# Autodesk Inventor assembly: Assembly1
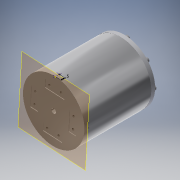
[picture p0: Inventor's stored thumbnail of the model, 180x180]
Saved by Autodesk Inventor 2017 (Build 210142000, 142)
## iProperties
Created: 2016-07-05
Part Number: Assembly1
Document SubType Name: Assembly
Designer: Andres
Author: Andres
## Documents named in this file (6)
- \\Mac\Home\Documents\repositorios\BoreholeCamera\CAD_Probe\Enclosure\Assembly\Assembly1.iam
- \\Mac\Home\Documents\repositorios\BoreholeCamera\CAD_Probe\Enclosure\Parts\Enclosure.ipt
- \\Mac\Home\Documents\repositorios\BoreholeCamera\CAD_Probe\Enclosure\Parts\TYPE 316 SS SOCKET HEAD CAP SCREW.ipt
- \\Mac\Home\Documents\repositorios\BoreholeCamera\CAD_Probe\Enclosure\Parts\SealCover.ipt
- \\Mac\Home\Documents\repositorios\BoreholeCamera\CAD_Probe\Enclosure\Assembly\Assembly1\Design Accelerator\O-Ring3.iam
- \\Mac\Home\Documents\repositorios\BoreholeCamera\CAD_Probe\Enclosure\Assembly\Cover.iam
## Components (13 placed, 5 different names)
1. Enclosure:1 — Rigid:1, Rigid:2, Mate:1, Mate:2, Rigid:3
2. Cover:2 [sub-assembly] — Rigid:3
3. TYPE 316 SS SOCKET HEAD CAP SCREW:2
4. TYPE 316 SS SOCKET HEAD CAP SCREW:4
5. TYPE 316 SS SOCKET HEAD CAP SCREW:6
6. TYPE 316 SS SOCKET HEAD CAP SCREW:7
7. TYPE 316 SS SOCKET HEAD CAP SCREW:8
8. TYPE 316 SS SOCKET HEAD CAP SCREW:9
9. TYPE 316 SS SOCKET HEAD CAP SCREW:11
10. TYPE 316 SS SOCKET HEAD CAP SCREW:12
11. SealCover:1 — Rigid:1
12. SealCover:2 — Rigid:2
13. O-Ring:1 [sub-assembly] — Mate:1, Mate:2
## Relationships (5: WeldJoint 3, Mate 2)
- Rigid:1 [WeldJoint]: Enclosure:1 ↔ SealCover:1
- Rigid:2 [WeldJoint]: Enclosure:1 ↔ SealCover:2
- Mate:1: Enclosure:1 ↔ O-Ring:1
- Mate:2: Enclosure:1 ↔ O-Ring:1
- Rigid:3 [WeldJoint]: Enclosure:1 ↔ Cover:2
